# Autodesk Inventor assembly: 16mm-LED-Power-Button
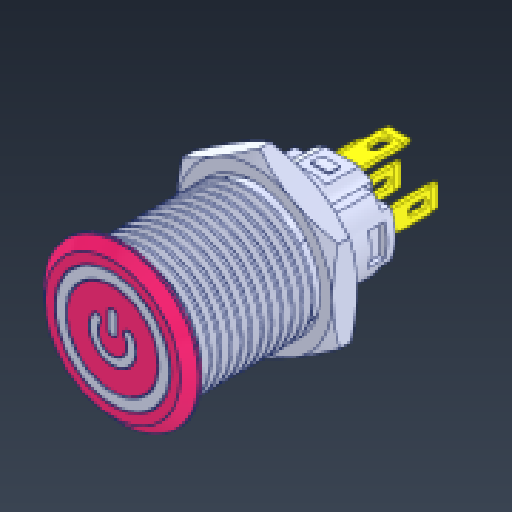
[picture p0: Inventor's stored thumbnail of the model, 512x512]
Saved by Autodesk Inventor 2023 (Build 270158000, 158)
## iProperties
Created: 2020-02-21
Part Number: 16mm-LED-Power-Button
Document SubType Name: Assembly
Designer: szymo
Sending System: SolidWorks 2019
Last Author: jswob
Last Saved: 2020-02-24
Author: szymo
## Documents named in this file (4)
- D:\tech\diy\e-skateboard\projekcik-inventor\buttoj\16mm-LED-Power-Button.iam
- D:\tech\diy\e-skateboard\projekcik-inventor\buttoj\Button_Body.ipt
- D:\tech\diy\e-skateboard\projekcik-inventor\buttoj\Socket.ipt
- D:\tech\diy\e-skateboard\projekcik-inventor\buttoj\Hex_Nut_M16-3mm.ipt
## Components (3 placed, 3 different names)
1. Button_Body:1 — Mate:1
2. Socket:1
3. Hex_Nut_M16-3mm:2 — Mate:1
## Relationships (1: Mate 1)
- Mate:1: Button_Body:1 ↔ Hex_Nut_M16-3mm:2
